# Autodesk Inventor assembly: Reactor Rod Holder Positions
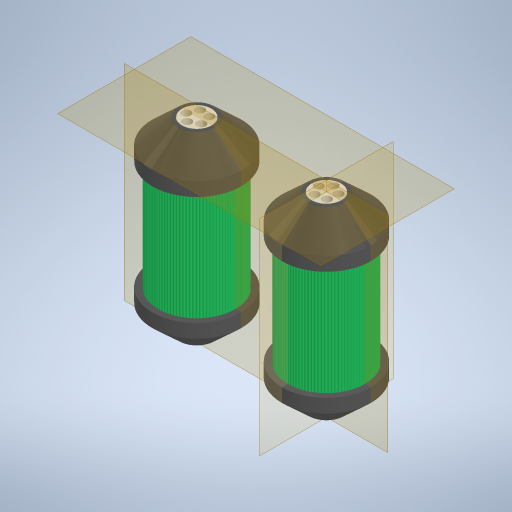
[picture p0: Inventor's stored thumbnail of the model, 512x512]
Saved by Autodesk Inventor 2024 (Build 280153020, 153B)
## iProperties
Created: 2023-08-02
Part Number: Reactor Rod Holder Positions
Document SubType Name: Assembly
Designer: torban
Author: torban
## Documents named in this file (2)
- D:\GIT\CIRC-2023-Night-Task-HW-SW\CAD\Reactor Module\Reactor Module\Reactor Rod Holder Positions.iam
- D:\GIT\CIRC-2023-Night-Task-HW-SW\CAD\Reactor Module\Reactor Module\Final.iam
## Components (2 placed, 1 different names)
1. Final:2 [sub-assembly] — Mate:3, Flush:1, Mate:5
2. Final:3 [sub-assembly] — Mate:3, Flush:1, Mate:4, Flush:2
## Relationships (5: Mate 3, Flush 2)
- Mate:3 (95 mm): Final:2 ↔ Final:3
- Flush:1: Final:2 ↔ Final:3
- Mate:4: Final:3
- Mate:5: Final:2
- Flush:2: Final:3
